# Autodesk Inventor assembly: pleuel_big
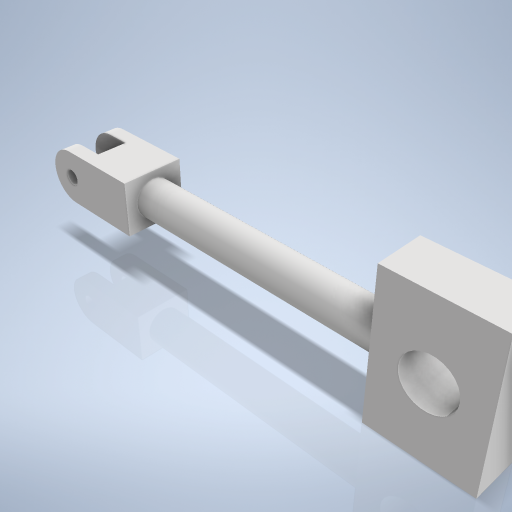
[picture p0: Inventor's stored thumbnail of the model, 512x512]
Saved by Autodesk Inventor 2024.2 (Build 282272000, 272)
## iProperties
Created: 2024-05-15
Part Number: pleuel_big
Document SubType Name: Assembly
Designer: Fabri
Author: Fabri
## Documents named in this file (3)
- C:\Users\Fabri\Documents\Inventor\Stirlingfan\pleuel_big.iam
- C:\Users\Fabri\Documents\Inventor\Stirlingfan\pleuel_m4.ipt
- C:\Users\Fabri\Documents\Inventor\Stirlingfan\25.ipt
## Components (2 placed, 2 different names)
1. pleuel_m4:1 — Einfügen:1
2. 25:1 — Einfügen:1
## Relationships (1: Insert 1)
- Einfügen:1 [Insert] (-5 mm): pleuel_m4:1 ↔ 25:1
